# Autodesk Inventor assembly: assembly of 13 and 2
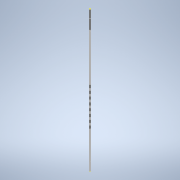
[picture p0: Inventor's stored thumbnail of the model, 180x180]
Saved by Autodesk Inventor 2020 (Build 240168000, 168)
## iProperties
Created: 2019-06-12
Part Number: assembly of 13 and 2
Document SubType Name: Weldment
Designer: ColinP
Weld Material: Welded Aluminum-6061
Mass: 1.42731 g
Surface Area: 47.5862 cm^2
Volume: 1.42731 cm^3
Density: 1 g/cm^3
Author: ColinP
## Documents named in this file (3)
- C:\Users\ColinP\Documents\Inventor\igor\assembly of 13 and 2.iam
- C:\Users\ColinP\Documents\Inventor\igor\burner_rod_1or3.ipt
- C:\Users\ColinP\Documents\Inventor\igor\burder_rod_2.ipt
## Components (3 placed, 2 different names)
1. burner_rod_1or3:1 — Insert:1
2. burder_rod_2:1 — Insert:1, Insert:2
3. burner_rod_1or3:2 — Insert:2
## Relationships (2: Insert 2)
- Insert:1: burner_rod_1or3:1 ↔ burder_rod_2:1
- Insert:2: burder_rod_2:1 ↔ burner_rod_1or3:2
